# Autodesk Inventor assembly: stemSectionBwithSphereAttachmentShape01
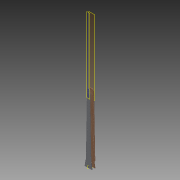
[picture p0: Inventor's stored thumbnail of the model, 180x180]
Saved by Autodesk Inventor 2013 (Build 170138000, 138)
## iProperties
Created: 2014-11-12
Part Number: stemSectionBwithSphereAttachmentShape01
Document SubType Name: Assembly
Designer: Nano
Author: Nano
## Documents named in this file (3)
- C:\Users\Nano\Documents\InventorByron\InventorMasterProject\octoBoto\stemSectionBwithSphereAttachmentShape01.iam
- C:\Users\Nano\Documents\InventorByron\InventorMasterProject\octoBoto\octoBotoStemSectC_v01.ipt
- C:\Users\Nano\Documents\InventorByron\InventorMasterProject\octoBoto\octoBotoStemRibSectB_v01.ipt
## Components (2 placed, 2 different names)
1. octoBotoStemSectC_v01:1 — Mate:1
2. octoBotoStemRibSectB_v01:1 — Mate:1
## Relationships (1: Mate 1)
- Mate:1: octoBotoStemSectC_v01:1 ↔ octoBotoStemRibSectB_v01:1
